# Autodesk Inventor assembly: Head
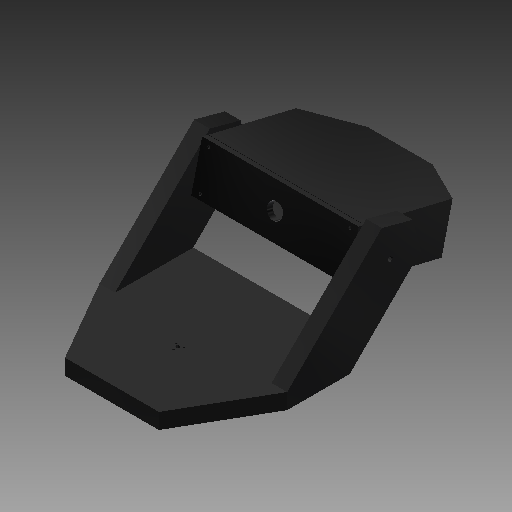
[picture p0: Inventor's stored thumbnail of the model, 512x512]
Saved by Autodesk Inventor 2017 (Build 210142000, 142)
## iProperties
Created: 2018-10-18
Part Number: Head
Document SubType Name: Assembly
Designer: Dell
Author: Dell
## Documents named in this file (6)
- C:\Users\Dell\Documents\GitHub\tr2\Head\Head.iam
- C:\Users\Dell\Documents\GitHub\tr2\Head\HA01.ipt
- C:\Users\Dell\Documents\GitHub\tr2\Head\Orbbec Astra\Orbbec Astra.iam
- C:\Users\Dell\Documents\GitHub\tr2\Head\HA02.ipt
- C:\Users\Dell\Documents\GitHub\tr2\Wheel Assembly\6mm Mounting Hub, thin.ipt
- C:\Users\Dell\Documents\GitHub\tr2\Head\HA03.ipt
## Components (5 placed, 5 different names)
1. HA01:1 — Mate:1, Flush:1, Mate:2, Mate:7, Mate:11, Mate:12, Mate:13
2. HA02:1 — Mate:2, Mate:4, Mate:5, Mate:6, Mate:7, Mate:8, Mate:9, Mate:10
3. HA03:1 — Mate:11, Mate:12, Mate:13
4. Orbbec Astra:1 [sub-assembly] — Mate:1, Flush:1
5. 6mm Mounting Hub, thin:1 — Mate:8, Mate:9, Mate:10
## Relationships (13: Mate 12, Flush 1)
- Mate:1 (2 mm): HA01:1 ↔ Orbbec Astra:1
- Flush:1 (-20 mm): HA01:1 ↔ Orbbec Astra:1
- Mate:2: HA01:1 ↔ HA02:1
- Mate:4: HA02:1
- Mate:5 (125 mm): HA02:1
- Mate:6: HA02:1
- Mate:7: HA01:1 ↔ HA02:1
- Mate:8: HA02:1 ↔ 6mm Mounting Hub, thin:1
- Mate:9: HA02:1 ↔ 6mm Mounting Hub, thin:1
- Mate:10: HA02:1 ↔ 6mm Mounting Hub, thin:1
- Mate:11: HA01:1 ↔ HA03:1
- Mate:12: HA01:1 ↔ HA03:1
- Mate:13: HA01:1 ↔ HA03:1
